# Autodesk Inventor assembly: motorizedSwitchHanger
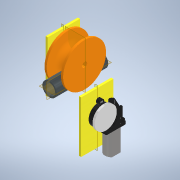
[picture p0: Inventor's stored thumbnail of the model, 180x180]
Saved by Autodesk Inventor 2020.2 (Build 242310000, 310)
## iProperties
Created: 2020-01-06
Part Number: motorizedSwitchHanger
Document SubType Name: Assembly
Designer: steele
Author: steele
## Documents named in this file (6)
- C:\git\CAD-Development\robSteele\2020 Lift Mechanism\motorizedSwitchHanger.iam
- C:\git\CAD-Development\robSteele\2020 Lift Mechanism\switchHangingPipe.ipt
- C:\git\CAD-Development\robSteele\2020 Lift Mechanism\wheelForHangingAndMoving.ipt
- C:\git\CAD-Development\robSteele\2020 Lift Mechanism\plateForHangingMechanism.ipt
- C:\git\CAD-Development\robSteele\2020 Lift Mechanism\am-2986 FR8ZZ Hex Bearing.ipt
- C:\git\CAD-Development\robSteele\2020 Lift Mechanism\am-2235a.iam
## Components (6 placed, 5 different names)
1. switchHangingPipe:1 — Flush:1, Flush:2, Flush:3
2. wheelForHangingAndMoving:1 — Flush:1, Flush:2, Flush:3, Insert:3, Mate:5
3. plateForHangingMechanism:1 — Insert:1, Insert:3, Mate:5
4. plateForHangingMechanism:2 — Insert:2
5. am-2986 FR8ZZ Hex Bearing:1 — Insert:1
6. am-2235a:1 [sub-assembly] — Insert:2
## Relationships (7: Flush 3, Insert 3, Mate 1)
- Flush:1: switchHangingPipe:1 ↔ wheelForHangingAndMoving:1
- Flush:2: switchHangingPipe:1 ↔ wheelForHangingAndMoving:1
- Flush:3 (38.1 mm): switchHangingPipe:1 ↔ wheelForHangingAndMoving:1
- Insert:1: plateForHangingMechanism:1 ↔ am-2986 FR8ZZ Hex Bearing:1
- Insert:2 (-6.477 mm): plateForHangingMechanism:2 ↔ am-2235a:1
- Insert:3 (6.35 mm): wheelForHangingAndMoving:1 ↔ plateForHangingMechanism:1
- Mate:5: wheelForHangingAndMoving:1 ↔ plateForHangingMechanism:1
